# Autodesk Inventor assembly: ASY Disk Micro filter
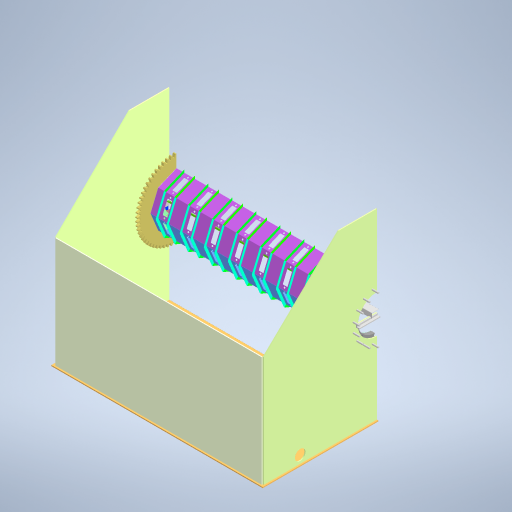
[picture p0: Inventor's stored thumbnail of the model, 512x512]
Saved by Autodesk Inventor 2024.2 (Build 282272000, 272)
## iProperties
Created: 2023-08-31
Part Number: ASY Disk Micro filter
Document SubType Name: Assembly
Designer: admin
Author: admin
## Documents named in this file (21)
- C:\Users\admin\YandexDisk-badmisterfox\домашниий пк\Inventor\DMF-Disk-Micro-Filter\ASY 000 ДМФ Disk Micro filter.iam
- C:\Users\admin\YandexDisk-badmisterfox\домашниий пк\Inventor\DMF-Disk-Micro-Filter\Left wall.ipt
- C:\Users\admin\YandexDisk-badmisterfox\домашниий пк\Inventor\DMF-Disk-Micro-Filter\Wall right.ipt
- C:\Users\admin\YandexDisk-badmisterfox\домашниий пк\Inventor\DMF-Disk-Micro-Filter\DF1.03 Wall bottom.ipt
- C:\Users\admin\YandexDisk-badmisterfox\домашниий пк\Inventor\DMF-Disk-Micro-Filter\DF1.04 Wall face.ipt
- C:\Users\admin\YandexDisk-badmisterfox\домашниий пк\Inventor\DMF-Disk-Micro-Filter\ыASY xDF frame.iam
- C:\Users\admin\YandexDisk-badmisterfox\домашниий пк\Inventor\DMF-Disk-Micro-Filter\ДМС 020 кольцо прижимное 1.ipt
- C:\Users\admin\YandexDisk-badmisterfox\домашниий пк\Inventor\DMF-Disk-Micro-Filter\ДМС 000 размеры.ipt
- C:\Users\admin\YandexDisk-badmisterfox\домашниий пк\Inventor\DMF-Disk-Micro-Filter\ASY ДМФ 100 кольцо со шпильками.iam
- C:\Users\admin\YandexDisk-badmisterfox\домашниий пк\Inventor\DMF-Disk-Micro-Filter\ДМС 040 лицо крышка.ipt
- C:\Users\admin\YandexDisk-badmisterfox\домашниий пк\Inventor\DMF-Disk-Micro-Filter\ASY ДМФ 0100 Барабан.iam
- C:\Users\admin\YandexDisk-badmisterfox\домашниий пк\Inventor\DMF-Disk-Micro-Filter\Постель 200 нос.ipt
- C:\Users\admin\YandexDisk-badmisterfox\домашниий пк\Inventor\DMF-Disk-Micro-Filter\ASY ДМФ 101 кольцо со шпильками зад.iam
- C:\Users\admin\YandexDisk-badmisterfox\домашниий пк\Inventor\DMF-Disk-Micro-Filter\ДМС 021 кольцо прижимное зад.ipt
- C:\Users\admin\YandexDisk-badmisterfox\домашниий пк\Inventor\DMF-Disk-Micro-Filter\Постель 201 зад.ipt
- C:\Users\admin\YandexDisk-badmisterfox\домашниий пк\Inventor\DMF-Disk-Micro-Filter\Постель 201 зад_CPY.ipt
- C:\Users\admin\YandexDisk-badmisterfox\домашниий пк\Inventor\DMF-Disk-Micro-Filter\ДМС 050 труба илоотвода.ipt
- C:\Users\admin\YandexDisk-badmisterfox\домашниий пк\Inventor\DMF-Disk-Micro-Filter\ДМС 045 держатель лотка.ipt
- C:\Users\admin\YandexDisk-badmisterfox\домашниий пк\Inventor\DMF-Disk-Micro-Filter\ДМС 053 усилитель кормовой 1.ipt
- C:\Users\admin\YandexDisk-badmisterfox\домашниий пк\Inventor\DMF-Disk-Micro-Filter\ASY ДМФ лоток 040 илоотвод.iam
- C:\Users\admin\YandexDisk-badmisterfox\домашниий пк\Inventor\DMF-Disk-Micro-Filter\Постель 200 нос_CPY.ipt
## Components (21 placed, 20 different names)
1. ДМС 000 размеры:1
2. Left wall:1 — Flush:3, Flush:4, Mate:1, Flush:6, Flush:7, Flush:9, Mate:4, Flush:16, Rotational:12, Rigid:9, Rigid:12
3. Wall right:1 — Flush:3, Mate:2, Flush:8, Flush:21, Rigid:6, Mate:22, Rotational:13
4. DF1.03 Wall bottom:1 — Mate:1, Mate:2, Flush:6, Flush:7, Flush:8, Mate:3, Flush:11, Mate:5
5. DF1.04 Wall face:1 — Flush:9, Mate:3, Mate:4, Flush:10
6. ASY DF frame:1 [sub-assembly] — Flush:15, Flush:13, Flush:14, Mate:5
7. ДМС 020 кольцо прижимное 1:1 — Rotational:12, Mate:13, Rotational:14
8. ASY ДМФ 100 кольцо со шпильками:1 [sub-assembly] — Flush:16, Rigid:9
9. ДМС 040 лицо крышка:1 — Mate:16, Rigid:8, Rigid:12
10. Постель 200 нос:2 — Flush:17, Rotational:14, Rigid:10, Rotational:15
11. Постель 200 нос_CPY:1 — Rigid:10
12. ASY ДМФ 0100 Барабан:1 [sub-assembly] — Rotational:15
13. ASY ДМФ 101 кольцо со шпильками зад:1 [sub-assembly] — Mate:14
14. ДМС 021 кольцо прижимное зад:1 — Flush:18, Rotational:13, Rigid:11
15. Постель 201 зад:1 — Mate:15, Rigid:3, Rigid:11
16. Постель 204 корма:1 — Rigid:3
17. ДМС 050 труба илоотвода:1 — Rigid:8, Tangent:1
18. ДМС 045 держатель лотка:1 — Mate:16, Mate:17, Tangent:1, Mate:23
19. ДМС 053 усилитель кормовой 1:1 — Flush:21, Rigid:6, Rigid:7
20. ДМС 053 усилитель кормовой 1:2 — Rigid:7
21. ASY ДМФ лоток 040 илоотвод:1 [sub-assembly] — Mate:22, Mate:23
## Relationships (42: Flush 16, Mate 13, WeldJoint 8, RevoluteJoint 4, Tangent 1)
- Flush:3: Left wall:1 ↔ Wall right:1
- Flush:4: Left wall:1
- Mate:1: Left wall:1 ↔ DF1.03 Wall bottom:1
- Mate:2: Wall right:1 ↔ DF1.03 Wall bottom:1
- Flush:6 (15 mm): Left wall:1 ↔ DF1.03 Wall bottom:1
- Flush:7 (25 mm): Left wall:1 ↔ DF1.03 Wall bottom:1
- Flush:8 (15 mm): Wall right:1 ↔ DF1.03 Wall bottom:1
- Flush:9: Left wall:1 ↔ DF1.04 Wall face:1
- Mate:3: DF1.03 Wall bottom:1 ↔ DF1.04 Wall face:1
- Mate:4: Left wall:1 ↔ DF1.04 Wall face:1
- Flush:10: DF1.04 Wall face:1
- Flush:11: DF1.03 Wall bottom:1
- [Flush]: ASY DF frame:1
- Flush:15: ASY DF frame:1
- Flush:13: ASY DF frame:1
- Flush:14: ASY DF frame:1
- Mate:5: DF1.03 Wall bottom:1 ↔ ASY DF frame:1
- Flush:16: Left wall:1 ↔ ASY ДМФ 100 кольцо со шпильками:1
- Rotational:12 [RevoluteJoint]: Left wall:1 ↔ ДМС 020 кольцо прижимное 1:1
- Mate:13: ДМС 020 кольцо прижимное 1:1
- Flush:17: Постель 200 нос:2
- Mate:14: ASY ДМФ 101 кольцо со шпильками зад:1
- Flush:18: ДМС 021 кольцо прижимное зад:1
- Mate:15: Постель 201 зад:1
- Rigid:3 [WeldJoint]: Постель 201 зад:1 ↔ Постель 204 корма:1
- [Mate]: ASY ДМФ лоток 040 илоотвод:1
- Mate:16: ДМС 040 лицо крышка:1 ↔ ДМС 045 держатель лотка:1
- Mate:17: ДМС 045 держатель лотка:1
- Flush:21: Wall right:1 ↔ ДМС 053 усилитель кормовой 1:1
- Rigid:6 [WeldJoint]: Wall right:1 ↔ ДМС 053 усилитель кормовой 1:1
- Rigid:7 [WeldJoint]: ДМС 053 усилитель кормовой 1:1 ↔ ДМС 053 усилитель кормовой 1:2
- Rigid:8 [WeldJoint]: ДМС 040 лицо крышка:1 ↔ ДМС 050 труба илоотвода:1
- Rigid:9 [WeldJoint]: Left wall:1 ↔ ASY ДМФ 100 кольцо со шпильками:1
- Tangent:1: ДМС 050 труба илоотвода:1 ↔ ДМС 045 держатель лотка:1
- Mate:22: Wall right:1 ↔ ASY ДМФ лоток 040 илоотвод:1
- Mate:23: ДМС 045 держатель лотка:1 ↔ ASY ДМФ лоток 040 илоотвод:1
- Rotational:13 [RevoluteJoint]: Wall right:1 ↔ ДМС 021 кольцо прижимное зад:1
- Rotational:14 [RevoluteJoint]: ДМС 020 кольцо прижимное 1:1 ↔ Постель 200 нос:2
- Rigid:10 [WeldJoint]: Постель 200 нос:2 ↔ Постель 200 нос_CPY:1
- Rotational:15 [RevoluteJoint]: Постель 200 нос:2 ↔ ASY ДМФ 0100 Барабан:1
- Rigid:11 [WeldJoint]: ДМС 021 кольцо прижимное зад:1 ↔ Постель 201 зад:1
- Rigid:12 [WeldJoint]: Left wall:1 ↔ ДМС 040 лицо крышка:1
